# Autodesk Inventor assembly: EngineAssemblyNEW
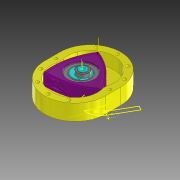
[picture p0: Inventor's stored thumbnail of the model, 180x180]
Saved by Autodesk Inventor 2020 (Build 240168000, 168)
## iProperties
Created: 2021-02-15
Part Number: EngineAssemblyNEW
Document SubType Name: Assembly
Designer: DDeGo
Author: DDeGo
## Documents named in this file (8)
- C:\Users\DDeGo\Documents\Drew\Projects\AirWankelEngine\cad\Wankel V2\EngineAssembly.iam
- C:\Users\DDeGo\Documents\Drew\Projects\AirWankelEngine\cad\Wankel V2\housing.ipt
- C:\Users\DDeGo\Documents\Drew\Projects\AirWankelEngine\cad\Wankel V2\housingPlate.ipt
- C:\Users\DDeGo\Documents\Drew\Projects\AirWankelEngine\cad\Wankel V2\piston.ipt
- C:\Users\DDeGo\Documents\Drew\Projects\AirWankelEngine\cad\hardware\6701 bearing.ipt
- C:\Users\DDeGo\Documents\Drew\Projects\AirWankelEngine\cad\hardware\MR85 bearing.ipt
- C:\Users\DDeGo\Documents\Drew\Projects\AirWankelEngine\cad\Wankel V2\camshaft.ipt
- C:\Users\DDeGo\Documents\Drew\Projects\AirWankelEngine\cad\hardware\ApexSeal_oring_2mm.ipt
## Components (10 placed, 7 different names)
1. housing:1 — Mate:9, Mate:10, Mate:14, Mate:15, Mate:16, Mate:17, Mate:44
2. housingPlate:1 — Mate:9, Mate:10, Mate:22, Mate:44
3. piston:1 — Mate:12, Mate:13, Mate:14, Rotation:1, Flush:5, Mate:41, Mate:42, Mate:43
4. 6701 bearing:1 — Mate:12, Mate:13, Mate:18
5. MR85 bearing:1 — Mate:15, Mate:16, Mate:19
6. camshaft:1 — Mate:17, Mate:18, Mate:19, Mate:21, Rotation:1
7. MR85 bearing:2 — Mate:21, Mate:22
8. ApexSeal_oring_2mm:1 — Flush:3, Flush:4, Flush:5, Mate:41
9. ApexSeal_oring_2mm:2 — Flush:3, Mate:42
10. ApexSeal_oring_2mm:3 — Flush:4, Mate:43
## Relationships (20: Mate 16, Flush 3, RelateRotation 1)
- Mate:9: housing:1 ↔ housingPlate:1
- Mate:10: housing:1 ↔ housingPlate:1
- Mate:12: piston:1 ↔ 6701 bearing:1
- Mate:13: piston:1 ↔ 6701 bearing:1
- Mate:14 (0.2 mm): housing:1 ↔ piston:1
- Mate:15: housing:1 ↔ MR85 bearing:1
- Mate:16: housing:1 ↔ MR85 bearing:1
- Mate:17: housing:1 ↔ camshaft:1
- Mate:18: 6701 bearing:1 ↔ camshaft:1
- Mate:19: MR85 bearing:1 ↔ camshaft:1
- Mate:21: camshaft:1 ↔ MR85 bearing:2
- Mate:22: housingPlate:1 ↔ MR85 bearing:2
- Rotation:1 [RelateRotation] (3 ul): piston:1 ↔ camshaft:1
- Flush:3: ApexSeal_oring_2mm:1 ↔ ApexSeal_oring_2mm:2
- Flush:4: ApexSeal_oring_2mm:1 ↔ ApexSeal_oring_2mm:3
- Flush:5: piston:1 ↔ ApexSeal_oring_2mm:1
- Mate:41: piston:1 ↔ ApexSeal_oring_2mm:1
- Mate:42: piston:1 ↔ ApexSeal_oring_2mm:2
- Mate:43: piston:1 ↔ ApexSeal_oring_2mm:3
- Mate:44: housing:1 ↔ housingPlate:1
